# Autodesk Inventor assembly: pullboxFiber
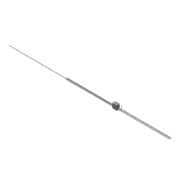
[picture p0: Inventor's stored thumbnail of the model, 180x180]
Saved by Autodesk Inventor 2016 (Build 200138000, 138)
## iProperties
Created: 2014-12-12
Part Number: pullboxFiber
Document SubType Name: Assembly
Designer: Dave
Author: Dave
## Documents named in this file (6)
- C:\Users\krosie\Google Drive\HERA\hera-cad\Node\pullboxFiber.iam
- C:\Users\krosie\Google Drive\HERA\hera-cad\Node\pullboxFiber.ipt
- C:\Users\krosie\Google Drive\HERA\hera-cad\Node\pipe_50mm_0.5m.ipt
- C:\Users\krosie\Google Drive\HERA\hera-cad\Node\sweep_50mm.ipt
- C:\Users\krosie\Google Drive\HERA\hera-cad\Node\pullboxFiberLid.ipt
- C:\Users\krosie\Google Drive\HERA\hera-cad\Node\pipe_50mm_Long.ipt
## Components (13 placed, 5 different names)
1. pullboxFiber:2 — Angle:1, Flush:1, Flush:2, Mate:1, Insert:6, Insert:7, Insert:8, Insert:9, Insert:10, Insert:11, Insert:12, Insert:13, Insert:14
2. pipe_50mm_0.5m:1 — Insert:5, Angle:1
3. pipe_50mm_0.5m:2 — Insert:4, Insert:6
4. sweep_50mm:1 — Insert:4, Insert:5
5. pullboxFiberLid:1 — Flush:1, Flush:2, Mate:1
6. pipe_50mm_Long:1 — Insert:7
7. pipe_50mm_Long:2 — Insert:8
8. pipe_50mm_Long:3 — Insert:9
9. pipe_50mm_Long:4 — Insert:11
10. pipe_50mm_Long:5 — Insert:12
11. pipe_50mm_Long:6 — Insert:10
12. pipe_50mm_Long:7 — Insert:14
13. pipe_50mm_Long:8 — Insert:13
## Relationships (15: Insert 11, Flush 2, Angle 1, Mate 1)
- Insert:4: pipe_50mm_0.5m:2 ↔ sweep_50mm:1
- Insert:5 (-101.6 mm): pipe_50mm_0.5m:1 ↔ sweep_50mm:1
- Angle:1 (180 deg): pullboxFiber:2 ↔ pipe_50mm_0.5m:1
- Flush:1: pullboxFiber:2 ↔ pullboxFiberLid:1
- Flush:2: pullboxFiber:2 ↔ pullboxFiberLid:1
- Mate:1 (5.08 mm): pullboxFiber:2 ↔ pullboxFiberLid:1
- Insert:6 (-254 mm): pullboxFiber:2 ↔ pipe_50mm_0.5m:2
- Insert:7 (-10000 mm): pullboxFiber:2 ↔ pipe_50mm_Long:1
- Insert:8 (-10000 mm): pullboxFiber:2 ↔ pipe_50mm_Long:2
- Insert:9 (-10000 mm): pullboxFiber:2 ↔ pipe_50mm_Long:3
- Insert:10 (-10000 mm): pullboxFiber:2 ↔ pipe_50mm_Long:6
- Insert:11 (-10000 mm): pullboxFiber:2 ↔ pipe_50mm_Long:4
- Insert:12 (-10000 mm): pullboxFiber:2 ↔ pipe_50mm_Long:5
- Insert:13: pullboxFiber:2 ↔ pipe_50mm_Long:8
- Insert:14: pullboxFiber:2 ↔ pipe_50mm_Long:7
